# Autodesk Inventor assembly: Baugruppe_Wetterstation
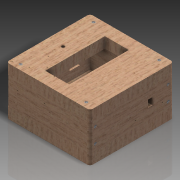
[picture p0: Inventor's stored thumbnail of the model, 180x180]
Saved by Autodesk Inventor 2014 SP1 (Build 180222100, 222)
## iProperties
Created: 2017-12-30
Part Number: Baugruppe_Wetterstation
Document SubType Name: Assembly
Designer: Flo
Author: Flo
## Documents named in this file (7)
- C:\Datenablage\Florian\Schule\NWT\GFS Wetterstation\Baugruppe_Wetterstation.iam
- C:\Datenablage\Florian\Schule\NWT\GFS Wetterstation\Seitenteil_mit_schalter.ipt
- C:\Datenablage\Florian\Schule\NWT\GFS Wetterstation\Seitenteil_mit_Sensoren.ipt
- C:\Datenablage\Florian\Schule\NWT\GFS Wetterstation\Seitenteil_links_rechts.ipt
- C:\Datenablage\Florian\Schule\NWT\GFS Wetterstation\Boden.ipt
- C:\Datenablage\Florian\Schule\NWT\GFS Wetterstation\Deckel.ipt
- C:\Datenablage\Florian\Schule\NWT\GFS Wetterstation\Wettterstation_Schraube.ipt
## Components (22 placed, 6 different names)
1. Seitenteil_mit_schalter:1 — Passend:1, Passend:2, Passend:3, Passend:4, Passend:10, Passend:13, Passend:32, Passend:33, Passend:34, Passend:35, Passend:36, Passend:37, Passend:38, Passend:39
2. Seitenteil_mit_Sensoren:1 — Passend:5, Passend:6, Passend:7, Passend:8, Passend:9, Passend:14, Passend:16, Passend:17, Passend:18, Passend:19, Passend:20, Passend:21, Passend:22, Passend:23
3. Seitenteil_links_rechts:1 — Passend:3, Passend:4, Passend:6, Passend:8, Passend:11
4. Seitenteil_links_rechts:2 — Passend:1, Passend:2, Passend:5, Passend:7, Passend:12, Passend:15
5. Boden:1 — Passend:9, Passend:10, Passend:11, Passend:40, Passend:41, Passend:42, Passend:43, Passend:44, Passend:45, Passend:46, Passend:47
6. Deckel:1 — Passend:12, Passend:13, Passend:14, Passend:15, Passend:24, Passend:25, Passend:26, Passend:27, Passend:28, Passend:29, Passend:30, Passend:31
7. Wettterstation_Schraube:1 — Passend:16, Passend:17
8. Wettterstation_Schraube:2 — Passend:18, Passend:19
9. Wettterstation_Schraube:3 — Passend:20, Passend:21
10. Wettterstation_Schraube:4 — Passend:22, Passend:23
11. Wettterstation_Schraube:5 — Passend:26, Passend:27
12. Wettterstation_Schraube:6 — Passend:24, Passend:25
13. Wettterstation_Schraube:7 — Passend:28, Passend:29
14. Wettterstation_Schraube:8 — Passend:30, Passend:31
15. Wettterstation_Schraube:9 — Passend:36, Passend:37
16. Wettterstation_Schraube:10 — Passend:38, Passend:39
17. Wettterstation_Schraube:11 — Passend:32, Passend:33
18. Wettterstation_Schraube:12 — Passend:34, Passend:35
19. Wettterstation_Schraube:13 — Passend:40, Passend:41
20. Wettterstation_Schraube:14 — Passend:42, Passend:43
21. Wettterstation_Schraube:15 — Passend:46, Passend:47
22. Wettterstation_Schraube:16 — Passend:44, Passend:45
## Relationships (47: Mate 47)
- Passend:1 [Mate]: Seitenteil_mit_schalter:1 ↔ Seitenteil_links_rechts:2
- Passend:2 [Mate]: Seitenteil_mit_schalter:1 ↔ Seitenteil_links_rechts:2
- Passend:3 [Mate]: Seitenteil_mit_schalter:1 ↔ Seitenteil_links_rechts:1
- Passend:4 [Mate]: Seitenteil_mit_schalter:1 ↔ Seitenteil_links_rechts:1
- Passend:5 [Mate]: Seitenteil_mit_Sensoren:1 ↔ Seitenteil_links_rechts:2
- Passend:6 [Mate]: Seitenteil_mit_Sensoren:1 ↔ Seitenteil_links_rechts:1
- Passend:7 [Mate]: Seitenteil_mit_Sensoren:1 ↔ Seitenteil_links_rechts:2
- Passend:8 [Mate]: Seitenteil_mit_Sensoren:1 ↔ Seitenteil_links_rechts:1
- Passend:9 [Mate]: Seitenteil_mit_Sensoren:1 ↔ Boden:1
- Passend:10 [Mate]: Seitenteil_mit_schalter:1 ↔ Boden:1
- Passend:11 [Mate]: Seitenteil_links_rechts:1 ↔ Boden:1
- Passend:12 [Mate]: Seitenteil_links_rechts:2 ↔ Deckel:1
- Passend:13 [Mate]: Seitenteil_mit_schalter:1 ↔ Deckel:1
- Passend:14 [Mate]: Seitenteil_mit_Sensoren:1 ↔ Deckel:1
- Passend:15 [Mate]: Seitenteil_links_rechts:2 ↔ Deckel:1
- Passend:16 [Mate]: Seitenteil_mit_Sensoren:1 ↔ Wettterstation_Schraube:1
- Passend:17 [Mate]: Seitenteil_mit_Sensoren:1 ↔ Wettterstation_Schraube:1
- Passend:18 [Mate]: Seitenteil_mit_Sensoren:1 ↔ Wettterstation_Schraube:2
- Passend:19 [Mate]: Seitenteil_mit_Sensoren:1 ↔ Wettterstation_Schraube:2
- Passend:20 [Mate]: Seitenteil_mit_Sensoren:1 ↔ Wettterstation_Schraube:3
- Passend:21 [Mate]: Seitenteil_mit_Sensoren:1 ↔ Wettterstation_Schraube:3
- Passend:22 [Mate]: Seitenteil_mit_Sensoren:1 ↔ Wettterstation_Schraube:4
- Passend:23 [Mate]: Seitenteil_mit_Sensoren:1 ↔ Wettterstation_Schraube:4
- Passend:24 [Mate]: Deckel:1 ↔ Wettterstation_Schraube:6
- Passend:25 [Mate]: Deckel:1 ↔ Wettterstation_Schraube:6
- Passend:26 [Mate]: Deckel:1 ↔ Wettterstation_Schraube:5
- Passend:27 [Mate]: Deckel:1 ↔ Wettterstation_Schraube:5
- Passend:28 [Mate]: Deckel:1 ↔ Wettterstation_Schraube:7
- Passend:29 [Mate]: Deckel:1 ↔ Wettterstation_Schraube:7
- Passend:30 [Mate]: Deckel:1 ↔ Wettterstation_Schraube:8
- Passend:31 [Mate]: Deckel:1 ↔ Wettterstation_Schraube:8
- Passend:32 [Mate]: Seitenteil_mit_schalter:1 ↔ Wettterstation_Schraube:11
- Passend:33 [Mate]: Seitenteil_mit_schalter:1 ↔ Wettterstation_Schraube:11
- Passend:34 [Mate]: Seitenteil_mit_schalter:1 ↔ Wettterstation_Schraube:12
- Passend:35 [Mate]: Seitenteil_mit_schalter:1 ↔ Wettterstation_Schraube:12
- Passend:36 [Mate]: Seitenteil_mit_schalter:1 ↔ Wettterstation_Schraube:9
- Passend:37 [Mate]: Seitenteil_mit_schalter:1 ↔ Wettterstation_Schraube:9
- Passend:38 [Mate]: Seitenteil_mit_schalter:1 ↔ Wettterstation_Schraube:10
- Passend:39 [Mate]: Seitenteil_mit_schalter:1 ↔ Wettterstation_Schraube:10
- Passend:40 [Mate]: Boden:1 ↔ Wettterstation_Schraube:13
- Passend:41 [Mate]: Boden:1 ↔ Wettterstation_Schraube:13
- Passend:42 [Mate]: Boden:1 ↔ Wettterstation_Schraube:14
- Passend:43 [Mate]: Boden:1 ↔ Wettterstation_Schraube:14
- Passend:44 [Mate]: Boden:1 ↔ Wettterstation_Schraube:16
- Passend:45 [Mate]: Boden:1 ↔ Wettterstation_Schraube:16
- Passend:46 [Mate]: Boden:1 ↔ Wettterstation_Schraube:15
- Passend:47 [Mate]: Boden:1 ↔ Wettterstation_Schraube:15
